# Autodesk Inventor assembly: Vane
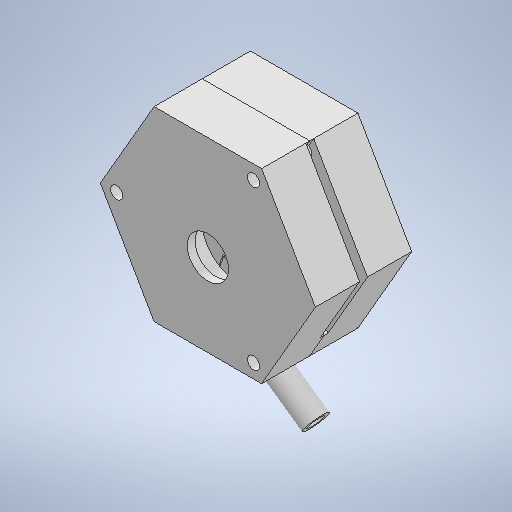
[picture p0: Inventor's stored thumbnail of the model, 512x512]
Saved by Autodesk Inventor 2026.1 (Build 301233020, 233B)
## iProperties
Created: 2025-10-21
Part Number: Vane
Document SubType Name: Assembly
Designer: yo
Author: yo
## Documents named in this file (6)
- C:\Users\yo\Documents\Andes\9no Semestre\Proyecto Intermedio\Proyecto\Huron-Hudson\Vane Engine\V4\Vane.iam
- C:\Users\yo\Documents\Andes\9no Semestre\Proyecto Intermedio\Proyecto\Huron-Hudson\Vane Engine\V4\Case.ipt
- C:\Users\yo\Documents\Andes\9no Semestre\Proyecto Intermedio\Proyecto\Huron-Hudson\Vane Engine\V4\Rotor.ipt
- C:\Users\yo\Documents\Andes\9no Semestre\Proyecto Intermedio\Proyecto\Huron-Hudson\Vane Engine\V4\Nozzle.ipt
- C:\Users\yo\Documents\Andes\9no Semestre\Proyecto Intermedio\Proyecto\Huron-Hudson\Vane Engine\V4\Vane.ipt
- C:\Users\yo\Documents\Andes\9no Semestre\Proyecto Intermedio\Proyecto\Huron-Hudson\Vane Engine\V4\Case_MIR.ipt
## Components (8 placed, 5 different names)
1. Case:1 — Flush:1, Flush:2, Flush:3, Mate:1, Mate:2, Mate:3, Flush:4, Tangent:1, Tangent:2, Tangent:3, Tangent:4, Mate:9, Mate:10
2. Rotor:1 — Mate:1, Mate:2, Mate:4, Mate:5, Mate:6, Mate:7, Flush:5, Flush:6, Flush:7, Flush:9, Mate:8
3. Nozzle:1 — Mate:3, Flush:4
4. Vane:1 — Mate:4, Tangent:1, Flush:6
5. Vane:2 — Mate:5, Tangent:2, Flush:7
6. Vane:3 — Mate:6, Tangent:3, Flush:5
7. Vane:4 — Mate:7, Tangent:4, Flush:9
8. Case_MIR:1 — Mate:8, Mate:9, Mate:10
## Relationships (22: Mate 10, Flush 8, Tangent 4)
- Flush:1: Case:1
- Flush:2: Case:1
- Flush:3: Case:1
- Mate:1: Case:1 ↔ Rotor:1
- Mate:2 (0.25 mm): Case:1 ↔ Rotor:1
- Mate:3: Case:1 ↔ Nozzle:1
- Flush:4: Case:1 ↔ Nozzle:1
- Mate:4 (0.2 mm): Rotor:1 ↔ Vane:1
- Tangent:1: Case:1 ↔ Vane:1
- Mate:5 (0.2 mm): Rotor:1 ↔ Vane:2
- Tangent:2: Case:1 ↔ Vane:2
- Mate:6 (0.2 mm): Rotor:1 ↔ Vane:3
- Tangent:3: Case:1 ↔ Vane:3
- Mate:7 (0.2 mm): Rotor:1 ↔ Vane:4
- Tangent:4: Case:1 ↔ Vane:4
- Flush:9: Rotor:1 ↔ Vane:4
- Flush:5: Rotor:1 ↔ Vane:3
- Flush:6: Rotor:1 ↔ Vane:1
- Flush:7: Rotor:1 ↔ Vane:2
- Mate:8: Rotor:1 ↔ Case_MIR:1
- Mate:9: Case:1 ↔ Case_MIR:1
- Mate:10: Case:1 ↔ Case_MIR:1
